# Autodesk Inventor assembly: Belt_Unit_Asem_Rev3
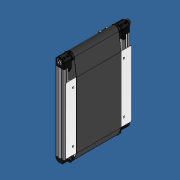
[picture p0: Inventor's stored thumbnail of the model, 180x180]
Saved by Autodesk Inventor 2020 (Build 240168000, 168)
## iProperties
Created: 2020-10-05
Part Number: Belt_Unit_Asem_Rev3
Document SubType Name: Assembly
Designer: kenta iguchi
Author: kenta iguchi
## Documents named in this file (29)
- D:\Document\Github\Cheap_Belt_Printer\Model\Asem\Belt_Unit_Asem_Rev3.iam
- D:\Document\Github\Cheap_Belt_Printer\Model\Parts\Bed_Parts\Bed Plate.ipt
- D:\Document\Github\Cheap_Belt_Printer\Model\Parts\Stepper Motor\NEMA17\Nema17_Geard\NEMA17_Geard.iam
- D:\Document\Github\Cheap_Belt_Printer\Model\Parts\MISUMI\FL6900ZZ_Autodesk_Inventor_2020_20201006\FL6900ZZ.ipt
- D:\Document\Github\Cheap_Belt_Printer\Model\Parts\Print_Parts\Print_Parts_L.ipt
- D:\Document\Github\Cheap_Belt_Printer\Model\Parts\Print_Parts\Print_Parts_N.ipt
- D:\Document\Github\Cheap_Belt_Printer\Model\Parts\Pulley\GT2\GT2_20t\GT2_20teeth_8bore.ipt
- D:\Document\Github\Cheap_Belt_Printer\Model\Parts\Shop_Parts\Φ35mm_Pipe.ipt
- D:\Document\Github\Cheap_Belt_Printer\Model\Parts\MISUMI\SSFRW10-230-MD6-N6_Autodesk_Inventor_2020_20201006\AIS2020\SSFRW10-230-MD6-N6_s.ipt
- D:\Document\Github\Cheap_Belt_Printer\Model\Parts\Bed_Parts\Build_Belt.ipt
- D:\Document\Github\Cheap_Belt_Printer\Model\Parts\Bed_Parts\Bed_Unit_Belt.ipt
- D:\Document\Github\Cheap_Belt_Printer\Model\Parts\MISUMI\HFS5-2020-270_Autodesk_Inventor_2020_20201011\HFS5-2020-270.ipt
- D:\Document\Github\Cheap_Belt_Printer\Model\Parts\Print_Parts\Rev2_Parts\Print_Parts_A1.ipt
- D:\Document\Github\Cheap_Belt_Printer\Model\Parts\MISUMI\SCCJ10-5_Autodesk_Inventor_2020_20201011\AIS2020\SCCJ10-5.iam
- D:\Document\Github\Cheap_Belt_Printer\Model\Parts\Print_Parts\Rev2_Parts\Print_Parts_A3.ipt
- D:\Document\Github\Cheap_Belt_Printer\Model\Parts\Print_Parts\Rev2_Parts\Print_Parts_A4.ipt
- D:\Document\Github\Cheap_Belt_Printer\Model\Parts\MISUMI\HFS5-2040-370_Autodesk_Inventor_2020_20201012\HFS5-2040-370.ipt
- D:\Document\Github\Cheap_Belt_Printer\Model\Parts\MISUMI\HBLFSNF5-SEC_Autodesk_Inventor_2020_20201031\AIS2020\HBLFSNF5-SEC_b.iam
- D:\Document\Github\Cheap_Belt_Printer\Model\Parts\MISUMI\HBLFSN5-SEC_Autodesk_Inventor_2020_20201031\AIS2020\HBLFSN5-SEC.iam
- D:\Document\Github\Cheap_Belt_Printer\Model\Parts\MISUMI\GPA32GT2060-A-P10_Autodesk_Inventor_2020_20201031\AIS2020\GPA32GT2060-A-P10.iam
- D:\Document\Github\Cheap_Belt_Printer\Model\Parts\Bolt\M4 x 10.ipt
- D:\Document\Github\Cheap_Belt_Printer\Model\Parts\Bolt\M3 x 15.ipt
- D:\Document\Github\Cheap_Belt_Printer\Model\Parts\Bolt\M5 x 45.ipt
- D:\Document\Github\Cheap_Belt_Printer\Model\Parts\Bolt\M4 x 20.ipt
- D:\Document\Github\Cheap_Belt_Printer\Model\Parts\Bolt\M5 x 35.ipt
- D:\Document\Github\Cheap_Belt_Printer\Model\Parts\Meviy\Belt_Unit_Motor_Holder.ipt
- D:\Document\Github\Cheap_Belt_Printer\Model\Parts\Meviy\Belt_Tenshon.ipt
- D:\Document\Github\Cheap_Belt_Printer\Model\Parts\MISUMI\SSFMRW10-234-M6-ND6_Autodesk_Inventor_2020_20210709\AIS2020\SSFMRW10-234-M6-ND6_s.ipt
- D:\Document\Github\Cheap_Belt_Printer\Model\Parts\MISUMI\SSFMR10-330_Autodesk_Inventor_2020_20210709\AIS2020\SSFMR10-330_s.ipt
## Components (67 placed, 28 different names)
1. Bed Plate:1 — メイト:13, Flush:33, Flush:38, Flush:39, Flush:43, Flush:44, Mate:47
2. Φ35mm_Pipe:1 — メイト:14, 挿入:22, Insert:29, Insert:30
3. Φ35mm_Pipe:2 — 挿入:23, Insert:40, Insert:41
4. FL6900ZZ:3 — Mate:30, 挿入:54, フラッシュ:56, 挿入:93
5. FL6900ZZ:4 — 挿入:94
6. Print_Parts_L:1 — メイト:13, 挿入:10, メイト:14, メイト:15, Mate:35, Insert:33, Flush:42, Insert:48, Insert:49, 挿入:69, 挿入:70
7. FL6900ZZ:6 — 挿入:10, Insert:38, メイト:71
8. Print_Parts_N:1 — メイト:15, Insert:38, 挿入:61, 挿入:62, 挿入:65, 挿入:66
9. SSFRW10-230-MD6-N6_s:1 — Mate:30, フラッシュ:56
10. Build_Belt:1 — 挿入:22, 挿入:23, Flush:33
11. Bed_Unit_Belt:1 — メイト:66, メイト:69, 挿入:92
12. FL6900ZZ:9 — Insert:35
13. FL6900ZZ:10 — Insert:34, Insert:39
14. HFS5-2020-270:1 — Flush:39, Mate:45, Flush:46, Mate:49, Mate:50, Flush:49, Flush:50, Mate:58, Mate:61
15. HFS5-2020-270:2 — Flush:38, Mate:46, Flush:47, Mate:48, Mate:51, Flush:48, Flush:51, Mate:56, Mate:62, Flush:55
16. Print_Parts_A1:1 — Insert:29
17. Print_Parts_A1:2 — Insert:30
18. Print_Parts_L:4 — Mate:35, Insert:34, Insert:35, Insert:36, Mate:36, Flush:42, Flush:43, Insert:46, 挿入:71, 挿入:72
19. FL6900ZZ:11 — Insert:33
20. Print_Parts_N:4 — Insert:36, Mate:36, 挿入:63, 挿入:64, 挿入:67, 挿入:68
21. SSFMR10-330_s:1 — メイト:70, メイト:71, 挿入:97, 挿入:98
22. SCCJ10-5:1 [sub-assembly] — Insert:39, 挿入:98
23. Print_Parts_A3:1 — Insert:40, 挿入:54
24. Print_Parts_A3:2 — Insert:41
25. Print_Parts_A4:1 — 挿入:95, メイト:72
26. HFS5-2040-370:1 — Insert:46, Mate:45, Flush:46, Mate:46, Flush:47, Mate:47, Mate:54, Mate:55, Mate:59, Mate:60, 挿入:95
27. HFS5-2040-370:2 — Insert:48, Insert:49, Flush:44, Insert:51, Insert:52, Mate:52, Mate:53, Mate:57, Mate:63, メイト:67, フラッシュ:57
28. NEMA17_Geard:3 [sub-assembly] — 挿入:87, メイト:69
29. Print_Parts_A4:2 — Insert:51, Insert:52, 挿入:83, 挿入:84
30. HBLFSNF5-SEC_b:1 [sub-assembly] — Mate:48, Mate:55, Flush:48
31. HBLFSNF5-SEC_b:2 [sub-assembly] — Mate:50, Mate:53, Flush:50
32. HBLFSNF5-SEC_b:3 [sub-assembly] — Mate:51, Mate:52, Flush:51
33. HBLFSNF5-SEC_b:4 [sub-assembly] — Mate:49, Mate:54, Flush:49
34. HBLFSN5-SEC:1 [sub-assembly] — Mate:56, Mate:57, Flush:52, Flush:53, Flush:55
35. HBLFSN5-SEC:2 [sub-assembly] — Mate:58, Mate:63, Flush:52
36. HBLFSN5-SEC:3 [sub-assembly] — Mate:60, Mate:61, Flush:54
37. HBLFSN5-SEC:4 [sub-assembly] — Mate:59, Mate:62, Flush:53, Flush:54
38. GPA32GT2060-A-P10:1 [sub-assembly] — メイト:66, メイト:70, 挿入:97
39. AS 1420 - Metric M4 x 10:1 — 挿入:86
40. AS 1420 - Metric M4 x 10:2 — 挿入:85
41. AS 1420 - Metric M3 x 15:1 — 挿入:91
42. AS 1420 - Metric M3 x 15:2 — 挿入:89
43. AS 1420 - Metric M3 x 15:3 — 挿入:90
44. AS 1420 - Metric M3 x 15:4 — 挿入:88
45. AS 1420 - Metric M5 x 45:1 — 挿入:62
46. AS 1420 - Metric M5 x 45:2 — 挿入:61
47. AS 1420 - Metric M5 x 45:3 — 挿入:63
48. AS 1420 - Metric M5 x 45:4 — 挿入:64
49. AS 1420 - Metric M4 x 20:1 — 挿入:66
50. AS 1420 - Metric M4 x 20:2 — 挿入:65
51. AS 1420 - Metric M4 x 20:3 — 挿入:67
52. AS 1420 - Metric M4 x 20:4 — 挿入:68
53. AS 1420 - Metric M4 x 10:3 — 挿入:72
54. AS 1420 - Metric M4 x 10:4 — 挿入:71
55. AS 1420 - Metric M4 x 10:5 — 挿入:70
56. AS 1420 - Metric M4 x 10:6 — 挿入:69
57. AS 1420 - Metric M4 x 10:7
58. AS 1420 - Metric M4 x 10:8
59. AS 1420 - Metric M4 x 10:9
60. AS 1420 - Metric M4 x 10:10
61. AS 1420 - Metric M5 x 35:3 — 挿入:83
62. AS 1420 - Metric M5 x 35:4 — 挿入:84
63. Belt_Unit_Motor_Holder:1 — メイト:67, フラッシュ:57, 挿入:85, 挿入:86, 挿入:87, 挿入:88, 挿入:89, 挿入:90, 挿入:91
64. GT2_20teeth_8bore:2 — 挿入:92
65. Belt_Tenshon:4 — 挿入:94, フラッシュ:58
66. Belt_Tenshon:5 — 挿入:93, フラッシュ:58, 挿入:96, メイト:72
67. SSFMRW10-234-M6-ND6_s:1 — 挿入:96
## Relationships (97: Insert 47, Mate 31, Flush 19)
- メイト:13 [Mate] (50 mm): Bed Plate:1 ↔ Print_Parts_L:1
- 挿入:10 [Insert]: Print_Parts_L:1 ↔ FL6900ZZ:6
- メイト:14 [Mate]: Φ35mm_Pipe:1 ↔ Print_Parts_L:1
- メイト:15 [Mate]: Print_Parts_L:1 ↔ Print_Parts_N:1
- 挿入:22 [Insert]: Φ35mm_Pipe:1 ↔ Build_Belt:1
- 挿入:23 [Insert]: Φ35mm_Pipe:2 ↔ Build_Belt:1
- Flush:33 (-50 mm): Bed Plate:1 ↔ Build_Belt:1
- Mate:30: FL6900ZZ:3 ↔ SSFRW10-230-MD6-N6_s:1
- Flush:38 (25 mm): Bed Plate:1 ↔ HFS5-2020-270:2
- Flush:39 (25 mm): Bed Plate:1 ↔ HFS5-2020-270:1
- Insert:29: Φ35mm_Pipe:1 ↔ Print_Parts_A1:1
- Insert:30: Φ35mm_Pipe:1 ↔ Print_Parts_A1:2
- Mate:35: Print_Parts_L:1 ↔ Print_Parts_L:4
- Insert:33: Print_Parts_L:1 ↔ FL6900ZZ:11
- Insert:34: FL6900ZZ:10 ↔ Print_Parts_L:4
- Insert:35: FL6900ZZ:9 ↔ Print_Parts_L:4
- Insert:36: Print_Parts_L:4 ↔ Print_Parts_N:4
- Mate:36: Print_Parts_L:4 ↔ Print_Parts_N:4
- Insert:38: FL6900ZZ:6 ↔ Print_Parts_N:1
- Insert:39: FL6900ZZ:10 ↔ SCCJ10-5:1
- Insert:40: Φ35mm_Pipe:2 ↔ Print_Parts_A3:1
- Insert:41: Φ35mm_Pipe:2 ↔ Print_Parts_A3:2
- Flush:42: Print_Parts_L:1 ↔ Print_Parts_L:4
- Flush:43: Bed Plate:1 ↔ Print_Parts_L:4
- Insert:46: Print_Parts_L:4 ↔ HFS5-2040-370:1
- Insert:48: Print_Parts_L:1 ↔ HFS5-2040-370:2
- Insert:49: Print_Parts_L:1 ↔ HFS5-2040-370:2
- Flush:44: Bed Plate:1 ↔ HFS5-2040-370:2
- Insert:51: HFS5-2040-370:2 ↔ Print_Parts_A4:2
- Insert:52: HFS5-2040-370:2 ↔ Print_Parts_A4:2
- Mate:45: HFS5-2020-270:1 ↔ HFS5-2040-370:1
- Flush:46: HFS5-2020-270:1 ↔ HFS5-2040-370:1
- Mate:46: HFS5-2020-270:2 ↔ HFS5-2040-370:1
- Flush:47: HFS5-2020-270:2 ↔ HFS5-2040-370:1
- Mate:47 (5 mm): Bed Plate:1 ↔ HFS5-2040-370:1
- Mate:48: HFS5-2020-270:2 ↔ HBLFSNF5-SEC_b:1
- Mate:49: HFS5-2020-270:1 ↔ HBLFSNF5-SEC_b:4
- Mate:50: HFS5-2020-270:1 ↔ HBLFSNF5-SEC_b:2
- Mate:51: HFS5-2020-270:2 ↔ HBLFSNF5-SEC_b:3
- Mate:52: HFS5-2040-370:2 ↔ HBLFSNF5-SEC_b:3
- Mate:53: HFS5-2040-370:2 ↔ HBLFSNF5-SEC_b:2
- Mate:54: HFS5-2040-370:1 ↔ HBLFSNF5-SEC_b:4
- Mate:55: HFS5-2040-370:1 ↔ HBLFSNF5-SEC_b:1
- Flush:48: HFS5-2020-270:2 ↔ HBLFSNF5-SEC_b:1
- Flush:49: HFS5-2020-270:1 ↔ HBLFSNF5-SEC_b:4
- Flush:50: HFS5-2020-270:1 ↔ HBLFSNF5-SEC_b:2
- Flush:51: HFS5-2020-270:2 ↔ HBLFSNF5-SEC_b:3
- Mate:56: HFS5-2020-270:2 ↔ HBLFSN5-SEC:1
- Mate:57: HFS5-2040-370:2 ↔ HBLFSN5-SEC:1
- Mate:58: HFS5-2020-270:1 ↔ HBLFSN5-SEC:2
- Mate:59: HFS5-2040-370:1 ↔ HBLFSN5-SEC:4
- Mate:60: HFS5-2040-370:1 ↔ HBLFSN5-SEC:3
- Mate:61: HFS5-2020-270:1 ↔ HBLFSN5-SEC:3
- Mate:62: HFS5-2020-270:2 ↔ HBLFSN5-SEC:4
- Mate:63: HFS5-2040-370:2 ↔ HBLFSN5-SEC:2
- Flush:52: HBLFSN5-SEC:1 ↔ HBLFSN5-SEC:2
- Flush:53: HBLFSN5-SEC:1 ↔ HBLFSN5-SEC:4
- Flush:54: HBLFSN5-SEC:3 ↔ HBLFSN5-SEC:4
- Flush:55: HFS5-2020-270:2 ↔ HBLFSN5-SEC:1
- 挿入:54 [Insert]: FL6900ZZ:3 ↔ Print_Parts_A3:1
- 挿入:61 [Insert]: Print_Parts_N:1 ↔ AS 1420 - Metric M5 x 45:2
- 挿入:62 [Insert]: Print_Parts_N:1 ↔ AS 1420 - Metric M5 x 45:1
- 挿入:63 [Insert]: Print_Parts_N:4 ↔ AS 1420 - Metric M5 x 45:3
- 挿入:64 [Insert]: Print_Parts_N:4 ↔ AS 1420 - Metric M5 x 45:4
- 挿入:65 [Insert]: Print_Parts_N:1 ↔ AS 1420 - Metric M4 x 20:2
- 挿入:66 [Insert]: Print_Parts_N:1 ↔ AS 1420 - Metric M4 x 20:1
- 挿入:67 [Insert]: Print_Parts_N:4 ↔ AS 1420 - Metric M4 x 20:3
- 挿入:68 [Insert]: Print_Parts_N:4 ↔ AS 1420 - Metric M4 x 20:4
- 挿入:69 [Insert]: Print_Parts_L:1 ↔ AS 1420 - Metric M4 x 10:6
- 挿入:70 [Insert]: Print_Parts_L:1 ↔ AS 1420 - Metric M4 x 10:5
- 挿入:71 [Insert]: Print_Parts_L:4 ↔ AS 1420 - Metric M4 x 10:4
- 挿入:72 [Insert]: Print_Parts_L:4 ↔ AS 1420 - Metric M4 x 10:3
- 挿入:83 [Insert]: Print_Parts_A4:2 ↔ AS 1420 - Metric M5 x 35:3
- 挿入:84 [Insert]: Print_Parts_A4:2 ↔ AS 1420 - Metric M5 x 35:4
- フラッシュ:56 [Flush] (-1.5 mm): FL6900ZZ:3 ↔ SSFRW10-230-MD6-N6_s:1
- メイト:66 [Mate]: Bed_Unit_Belt:1 ↔ GPA32GT2060-A-P10:1
- メイト:67 [Mate]: HFS5-2040-370:2 ↔ Belt_Unit_Motor_Holder:1
- フラッシュ:57 [Flush]: HFS5-2040-370:2 ↔ Belt_Unit_Motor_Holder:1
- 挿入:85 [Insert]: AS 1420 - Metric M4 x 10:2 ↔ Belt_Unit_Motor_Holder:1
- 挿入:86 [Insert]: AS 1420 - Metric M4 x 10:1 ↔ Belt_Unit_Motor_Holder:1
- 挿入:87 [Insert]: NEMA17_Geard:3 ↔ Belt_Unit_Motor_Holder:1
- 挿入:88 [Insert]: AS 1420 - Metric M3 x 15:4 ↔ Belt_Unit_Motor_Holder:1
- 挿入:89 [Insert]: AS 1420 - Metric M3 x 15:2 ↔ Belt_Unit_Motor_Holder:1
- 挿入:90 [Insert]: AS 1420 - Metric M3 x 15:3 ↔ Belt_Unit_Motor_Holder:1
- 挿入:91 [Insert]: AS 1420 - Metric M3 x 15:1 ↔ Belt_Unit_Motor_Holder:1
- メイト:69 [Mate]: Bed_Unit_Belt:1 ↔ NEMA17_Geard:3
- 挿入:92 [Insert] (1 mm): Bed_Unit_Belt:1 ↔ GT2_20teeth_8bore:2
- 挿入:93 [Insert] (0.5 mm): FL6900ZZ:3 ↔ Belt_Tenshon:5
- 挿入:94 [Insert] (0.5 mm): FL6900ZZ:4 ↔ Belt_Tenshon:4
- フラッシュ:58 [Flush]: Belt_Tenshon:4 ↔ Belt_Tenshon:5
- 挿入:95 [Insert]: Print_Parts_A4:1 ↔ HFS5-2040-370:1
- 挿入:96 [Insert]: Belt_Tenshon:5 ↔ SSFMRW10-234-M6-ND6_s:1
- メイト:70 [Mate]: SSFMR10-330_s:1 ↔ GPA32GT2060-A-P10:1
- メイト:71 [Mate]: FL6900ZZ:6 ↔ SSFMR10-330_s:1
- 挿入:97 [Insert]: SSFMR10-330_s:1 ↔ GPA32GT2060-A-P10:1
- 挿入:98 [Insert]: SSFMR10-330_s:1 ↔ SCCJ10-5:1
- メイト:72 [Mate]: Print_Parts_A4:1 ↔ Belt_Tenshon:5
